# Autodesk Inventor assembly: Skateboard Remote
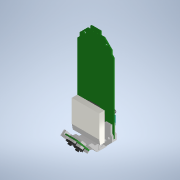
[picture p0: Inventor's stored thumbnail of the model, 180x180]
Saved by Autodesk Inventor 2020 (Build 240168000, 168)
## iProperties
Created: 2021-01-14
Part Number: Skateboard Remote
Document SubType Name: Assembly
Designer: Luke
Author: Luke
## Documents named in this file (9)
- C:\Users\Luke\Documents\Git Projects\Electric Skateboard V2\Part Files\Remote Parts\Skateboard Remote Smaller Angle Buttons.iam
- C:\Users\Luke\Documents\Git Projects\Electric Skateboard V2\Part Files\Remote Parts\PCB.ipt
- C:\Users\Luke\Documents\Git Projects\Electric Skateboard V2\Part Files\Remote Parts\Battery Spacer.ipt
- C:\Users\Luke\Documents\Git Projects\Electric Skateboard V2\Part Files\Remote Parts\Battery.ipt
- C:\Users\Luke\Documents\Git Projects\Electric Skateboard V2\Part Files\Remote Parts\Button Module.ipt
- C:\Users\Luke\Documents\Git Projects\Electric Skateboard V2\Part Files\Remote Parts\Joystick.ipt
- C:\Users\Luke\Documents\Git Projects\Electric Skateboard V2\Part Files\Remote Parts\Button.ipt
- C:\Users\Luke\Documents\Git Projects\Electric Skateboard V2\Part Files\Remote Parts\Button Holder Better Angle Top.ipt
- C:\Users\Luke\Documents\Git Projects\Electric Skateboard V2\Part Files\Remote Parts\Button Holder Bottom Smaller Angle.ipt
## Components (9 placed, 8 different names)
1. PCB:1 — Mate:1, Flush:1, Flush:2, Mate:2, Flush:6, Flush:8, Flush:9, Flush:10, Mate:14, Mate:15, Mate:16, Mate:24, Flush:12
2. Battery Spacer:1 — Mate:1, Flush:1, Flush:2, Flush:3
3. Battery:1 — Flush:3, Mate:2, Flush:12
4. Button Module:1 — Mate:6, Mate:7, Mate:8, Mate:9, Mate:10, Mate:11, Mate:22, Mate:23, Flush:11
5. Joystick:1 — Flush:6, Flush:8, Flush:9, Flush:10
6. Button:2 — Mate:6, Mate:7, Mate:8
7. Button:3 — Mate:9, Mate:10, Mate:11
8. Button Holder Better Angle Top:1 — Mate:14, Mate:15, Mate:16, Mate:20, Mate:21
9. Button Holder Bottom Smaller Angle:1 — Mate:20, Mate:21, Mate:22, Mate:23, Flush:11, Mate:24
## Relationships (25: Mate 16, Flush 9)
- Mate:1: PCB:1 ↔ Battery Spacer:1
- Flush:1 (9.27 mm): PCB:1 ↔ Battery Spacer:1
- Flush:2 (6.4 mm): PCB:1 ↔ Battery Spacer:1
- Flush:3: Battery Spacer:1 ↔ Battery:1
- Mate:2: PCB:1 ↔ Battery:1
- Flush:6: PCB:1 ↔ Joystick:1
- Flush:8: PCB:1 ↔ Joystick:1
- Flush:9: PCB:1 ↔ Joystick:1
- Flush:10: PCB:1 ↔ Joystick:1
- Mate:6: Button Module:1 ↔ Button:2
- Mate:7: Button Module:1 ↔ Button:2
- Mate:8: Button Module:1 ↔ Button:2
- Mate:9: Button Module:1 ↔ Button:3
- Mate:10: Button Module:1 ↔ Button:3
- Mate:11: Button Module:1 ↔ Button:3
- Mate:14: PCB:1 ↔ Button Holder Better Angle Top:1
- Mate:15: PCB:1 ↔ Button Holder Better Angle Top:1
- Mate:16: PCB:1 ↔ Button Holder Better Angle Top:1
- Mate:20: Button Holder Better Angle Top:1 ↔ Button Holder Bottom Smaller Angle:1
- Mate:21: Button Holder Better Angle Top:1 ↔ Button Holder Bottom Smaller Angle:1
- Mate:22: Button Module:1 ↔ Button Holder Bottom Smaller Angle:1
- Mate:23: Button Module:1 ↔ Button Holder Bottom Smaller Angle:1
- Flush:11: Button Module:1 ↔ Button Holder Bottom Smaller Angle:1
- Mate:24: PCB:1 ↔ Button Holder Bottom Smaller Angle:1
- Flush:12 (4 mm): PCB:1 ↔ Battery:1
